# Autodesk Inventor assembly: cornerFrame
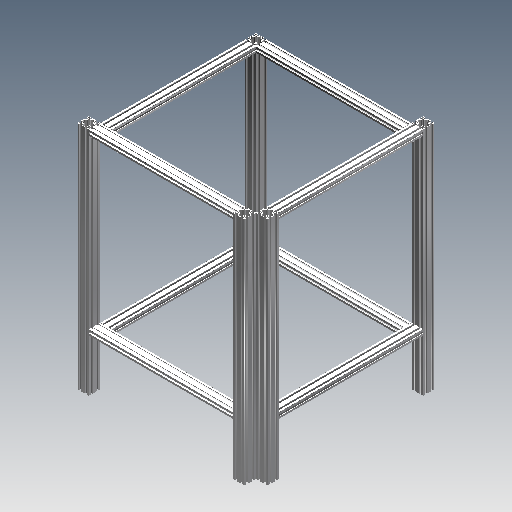
[picture p0: Inventor's stored thumbnail of the model, 512x512]
Saved by Autodesk Inventor 2018 (Build 220112000, 112)
## iProperties
Created: 2018-01-07
Part Number: cornerFrame
Document SubType Name: Assembly
Designer: sawaiz
Author: sawaiz
## Documents named in this file (4)
- C:\Users\sawaiz\OneDrive\projects\larkspurKitchen\frame\cornerFrame.iam
- C:\Users\sawaiz\OneDrive\projects\larkspurKitchen\frame\extrusions\HFS5-4040-800.ipt
- C:\Users\sawaiz\OneDrive\projects\larkspurKitchen\frame\plate.iam
- C:\Users\sawaiz\OneDrive\projects\larkspurKitchen\frame\extrusions\HFS5-2040-500.ipt
## Components (7 placed, 3 different names)
1. HFS5-4040-800:3 — Mate:4, Mate:5, Flush:12, Flush:16, Flush:17, Flush:18, Flush:19, Flush:20, Mate:8, Mate:9
2. HFS5-2040-500:1 — Mate:5, Flush:12, Flush:13, Flush:15, Flush:17, Mate:11
3. HFS5-2040-500:2 — Mate:4, Flush:13, Flush:16, Mate:10
4. HFS5-2040-500:3 — Flush:18, Flush:20, Mate:8, Flush:21
5. HFS5-2040-500:4 — Flush:19, Mate:9, Flush:21, Flush:22
6. plate:1 [sub-assembly] — Flush:14, Angle:1, Mate:6, Mate:7, Flush:22, Mate:10
7. plate:2 [sub-assembly] — Flush:14, Angle:1, Mate:6, Mate:7, Flush:15, Mate:11
## Relationships (20: Flush 11, Mate 8, Angle 1)
- Mate:4: HFS5-4040-800:3 ↔ HFS5-2040-500:2
- Mate:5: HFS5-4040-800:3 ↔ HFS5-2040-500:1
- Flush:12: HFS5-4040-800:3 ↔ HFS5-2040-500:1
- Flush:13: HFS5-2040-500:1 ↔ HFS5-2040-500:2
- Flush:14: plate:1 ↔ plate:2
- Angle:1 (90 deg): plate:1 ↔ plate:2
- Mate:6: plate:1 ↔ plate:2
- Mate:7: plate:1 ↔ plate:2
- Flush:15: HFS5-2040-500:1 ↔ plate:2
- Flush:16: HFS5-4040-800:3 ↔ HFS5-2040-500:2
- Flush:17: HFS5-4040-800:3 ↔ HFS5-2040-500:1
- Flush:18: HFS5-4040-800:3 ↔ HFS5-2040-500:3
- Flush:19: HFS5-4040-800:3 ↔ HFS5-2040-500:4
- Flush:20: HFS5-4040-800:3 ↔ HFS5-2040-500:3
- Mate:8: HFS5-4040-800:3 ↔ HFS5-2040-500:3
- Mate:9: HFS5-4040-800:3 ↔ HFS5-2040-500:4
- Flush:21: HFS5-2040-500:3 ↔ HFS5-2040-500:4
- Flush:22: HFS5-2040-500:4 ↔ plate:1
- Mate:10: HFS5-2040-500:2 ↔ plate:1
- Mate:11: HFS5-2040-500:1 ↔ plate:2
